# Autodesk Inventor assembly: assembly
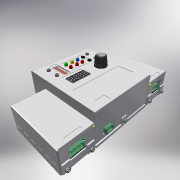
[picture p0: Inventor's stored thumbnail of the model, 180x180]
Saved by Autodesk Inventor 2019 (Build 230136000, 136)
## iProperties
Created: 2020-05-08
Part Number: assembly
Document SubType Name: Assembly
Designer: Mateusz
Author: Mateusz
## Documents named in this file (13)
- D:\Projekty\Azure Sphere IoT Controller\Controller\case\assembly.iam
- D:\Projekty\Azure Sphere IoT Controller\Controller\case\case_top.ipt
- D:\Projekty\Azure Sphere IoT Controller\Controller\case\electronic_holder.ipt
- D:\Projekty\Azure Sphere IoT Controller\Controller\case\case_bottom.ipt
- D:\Projekty\Azure Sphere IoT Controller\Controller\case\panel.iam
- D:\Projekty\Azure Sphere IoT Controller\Controller\case\4Digit_7Segment_LED_Display v8.ipt
- D:\Projekty\Azure Sphere IoT Controller\Controller\case\Turn knob.ipt
- D:\Projekty\Azure Sphere IoT Controller\Controller\case\SHCS M3-20.ipt
- D:\Projekty\Azure Sphere IoT Controller\Addons\Output\case\output_assembly.iam
- D:\Projekty\Azure Sphere IoT Controller\Controller\case\board.ipt
- D:\Projekty\Azure Sphere IoT Controller\Addons\Input\case\input_assembly.iam
- D:\Projekty\Azure Sphere IoT Controller\Controller\case\DIN_mount.ipt
- D:\Projekty\Azure Sphere IoT Controller\Controller\case\button.ipt
## Components (20 placed, 12 different names)
1. case_top:1 — Mate:3, Flush:1, Mate:4, Mate:5, Mate:6, Flush:2, Mate:12, Mate:13, Mate:14, Mate:15, Mate:16, Mate:17, Mate:18, Mate:19, Mate:20, Mate:21, Mate:22, Mate:23, Flush:4, Flush:7, Flush:8, Flush:10
2. electronic_holder:1 — Mate:3, Flush:1, Mate:4, Mate:7, Mate:8, Mate:9, Mate:30, Mate:31, Flush:5
3. case_bottom:1 — Mate:5, Mate:6, Flush:2, Mate:24, Mate:25, Mate:26, Mate:27, Mate:28, Mate:29, Mate:34, Mate:35, Mate:36, Mate:37, Mate:38, Mate:39
4. panel:1 [sub-assembly] — Mate:7, Mate:8, Mate:9, Mate:40, Mate:41, Mate:42, Mate:43
5. 4Digit_7Segment_LED_Display v8:1 — Mate:12, Mate:13, Flush:7
6. Turn knob:1 — Mate:14, Mate:15
7. SHCS M3-20:1 — Mate:20, Mate:21
8. SHCS M3-20:2 — Mate:22, Mate:23
9. SHCS M3-20:3 — Mate:16, Mate:17
10. SHCS M3-20:4 — Mate:18, Mate:19
11. SHCS M3-20:5 — Mate:24, Mate:28
12. SHCS M3-20:6 — Mate:25, Mate:27
13. SHCS M3-20:7 — Mate:26, Mate:29
14. output_assembly:1 [sub-assembly] — Flush:4, Mate:32, Flush:6
15. board:1 — Mate:30, Mate:31, Flush:5, Mate:32, Flush:6, Mate:33, Flush:9
16. input_assembly:1 [sub-assembly] — Flush:8, Mate:33, Flush:9
17. DIN_mount:1 — Mate:34, Mate:36, Mate:37
18. DIN_mount:2 — Mate:35, Mate:38, Mate:39
19. button:1 — Mate:42, Mate:43
20. button:2 — Mate:40, Mate:41
## Relationships (48: Mate 39, Flush 9)
- Mate:3: case_top:1 ↔ electronic_holder:1
- Flush:1: case_top:1 ↔ electronic_holder:1
- Mate:4 (0.5 mm): case_top:1 ↔ electronic_holder:1
- Mate:5: case_top:1 ↔ case_bottom:1
- Mate:6: case_top:1 ↔ case_bottom:1
- Flush:2: case_top:1 ↔ case_bottom:1
- Mate:7: electronic_holder:1 ↔ panel:1
- Mate:8: electronic_holder:1 ↔ panel:1
- Mate:9: electronic_holder:1 ↔ panel:1
- Mate:12 (0.5 mm): case_top:1 ↔ 4Digit_7Segment_LED_Display v8:1
- Mate:13: case_top:1 ↔ 4Digit_7Segment_LED_Display v8:1
- Mate:14: case_top:1 ↔ Turn knob:1
- Mate:15: case_top:1 ↔ Turn knob:1
- Mate:16: case_top:1 ↔ SHCS M3-20:3
- Mate:17: case_top:1 ↔ SHCS M3-20:3
- Mate:18: case_top:1 ↔ SHCS M3-20:4
- Mate:19: case_top:1 ↔ SHCS M3-20:4
- Mate:20: case_top:1 ↔ SHCS M3-20:1
- Mate:21: case_top:1 ↔ SHCS M3-20:1
- Mate:22: case_top:1 ↔ SHCS M3-20:2
- Mate:23: case_top:1 ↔ SHCS M3-20:2
- Mate:24: case_bottom:1 ↔ SHCS M3-20:5
- Mate:25: case_bottom:1 ↔ SHCS M3-20:6
- Mate:26: case_bottom:1 ↔ SHCS M3-20:7
- Mate:27: case_bottom:1 ↔ SHCS M3-20:6
- Mate:28: case_bottom:1 ↔ SHCS M3-20:5
- Mate:29: case_bottom:1 ↔ SHCS M3-20:7
- Flush:4: case_top:1 ↔ output_assembly:1
- Mate:30: electronic_holder:1 ↔ board:1
- Mate:31: electronic_holder:1 ↔ board:1
- Flush:5: electronic_holder:1 ↔ board:1
- Mate:32: output_assembly:1 ↔ board:1
- Flush:6: output_assembly:1 ↔ board:1
- Flush:7 (-1 mm): case_top:1 ↔ 4Digit_7Segment_LED_Display v8:1
- Flush:8: case_top:1 ↔ input_assembly:1
- Mate:33: board:1 ↔ input_assembly:1
- Flush:9: board:1 ↔ input_assembly:1
- Flush:10: case_top:1
- Mate:34: case_bottom:1 ↔ DIN_mount:1
- Mate:35: case_bottom:1 ↔ DIN_mount:2
- Mate:36: case_bottom:1 ↔ DIN_mount:1
- Mate:37: case_bottom:1 ↔ DIN_mount:1
- Mate:38: case_bottom:1 ↔ DIN_mount:2
- Mate:39: case_bottom:1 ↔ DIN_mount:2
- Mate:40: panel:1 ↔ button:2
- Mate:41 (0.5 mm): panel:1 ↔ button:2
- Mate:42: panel:1 ↔ button:1
- Mate:43 (0.5 mm): panel:1 ↔ button:1
